# Autodesk Inventor assembly: ASY GBK 3110 central wall shield 1
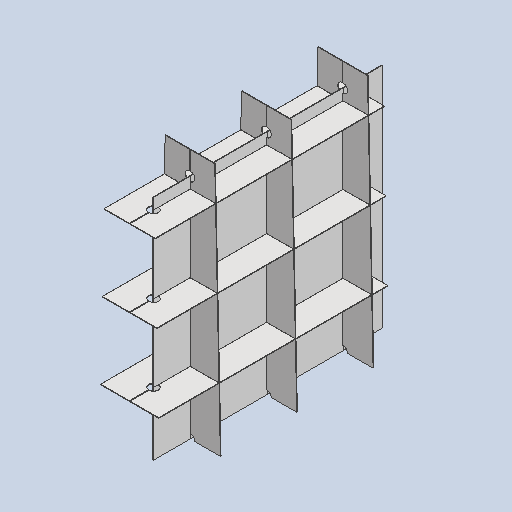
[picture p0: Inventor's stored thumbnail of the model, 512x512]
Saved by Autodesk Inventor 2026 (Build 300175000, 175)
## iProperties
Created: 2026-05-19
Part Number: ASY GBK 3110 central wall shield 1
Document SubType Name: Assembly
Designer: pokla
Mass: 174041 g
Surface Area: 113034 cm^2
Volume: 22170.8 cm^3
Density: 7.85 g/cm^3
Author: admin
## Documents named in this file (7)
- C:\Users\pokla\Documents\Inventor\GBK-Gubkinskiy\ASY GBK 3110 central wall shield 1.iam
- C:\Users\pokla\Documents\Inventor\GBK-Gubkinskiy\GBK 3113 stringer 1.ipt
- C:\Users\pokla\Documents\Inventor\GBK-Gubkinskiy\GBK 3111 shield 1.ipt
- C:\Users\pokla\Documents\Inventor\GBK-Gubkinskiy\GBK 3114 stringer 2.ipt
- C:\Users\pokla\Documents\Inventor\GBK-Gubkinskiy\GBK 3115 stringer 3.ipt
- C:\Users\pokla\Documents\Inventor\GBK-Gubkinskiy\GBK 3112 central main rib.ipt
- C:\Users\pokla\Documents\Inventor\GBK-Gubkinskiy\GBK 0101 main rib.ipt
## Components (13 placed, 8 different names)
1. GBK 3113 stringer 1.ipt:1 — Жесткий:1
2. GBK 3111 shield 1.ipt:1 — Заподлицо:5, Совмещение:5, Заподлицо:3, Совмещение:2, Заподлицо:1, Совмещение:1, Совмещение:4, Заподлицо:2
3. GBK 3114 stringer 2.ipt:1 — Жесткий:2
4. GBK 3115 stringer 3.ipt:1 — Жесткий:3
5. GBK 3113 stringer 1.ipt:2 — Жесткий:6
6. GBK 3114 stringer 2:3 — Жесткий:5
7. GBK 3115 stringer 3:2 — Жесткий:6
8. GBK 3112 central main rib.ipt:2 — Заподлицо:4, Совмещение:4, Заподлицо:2, Жесткий:6, Жесткий:5, Жесткий:6
9. GBK 3112 central main rib:3
10. GBK 3112 central main rib:4
11. GBK 3112 central main rib.ipt:1 — Заподлицо:5, Совмещение:5, Заподлицо:3, Заподлицо:4, Жесткий:1, Жесткий:2, Жесткий:3
12. GBK 3112 central main rib:5
13. GBK 3112 central main rib:6
## Component patterns: (3 elements, first: GBK 3112 central main rib.ipt:2), (3 elements, first: GBK 3112 central main rib.ipt:1)
## Relationships (15: WeldJoint 6, Flush 5, Mate 4)
- Заподлицо:5 [Flush] (254 mm): GBK 3111 shield 1.ipt:1 ↔ GBK 3112 central main rib.ipt:1
- Совмещение:5 [Mate]: GBK 3111 shield 1.ipt:1 ↔ GBK 3112 central main rib.ipt:1
- Заподлицо:3 [Flush]: GBK 3111 shield 1.ipt:1 ↔ GBK 3112 central main rib.ipt:1
- Совмещение:2 [Mate]: GBK 3111 shield 1.ipt:1
- Заподлицо:1 [Flush]: GBK 3111 shield 1.ipt:1
- Совмещение:1 [Mate]: GBK 3111 shield 1.ipt:1
- Заподлицо:4 [Flush]: GBK 3112 central main rib.ipt:2 ↔ GBK 3112 central main rib.ipt:1
- Совмещение:4 [Mate]: GBK 3111 shield 1.ipt:1 ↔ GBK 3112 central main rib.ipt:2
- Заподлицо:2 [Flush]: GBK 3111 shield 1.ipt:1 ↔ GBK 3112 central main rib.ipt:2
- Жесткий:1 [WeldJoint] (4 mm): GBK 3113 stringer 1.ipt:1 ↔ GBK 3112 central main rib.ipt:1
- Жесткий:2 [WeldJoint] (4 mm): GBK 3114 stringer 2.ipt:1 ↔ GBK 3112 central main rib.ipt:1
- Жесткий:3 [WeldJoint] (4 mm): GBK 3115 stringer 3.ipt:1 ↔ GBK 3112 central main rib.ipt:1
- Жесткий:6 [WeldJoint] (4 mm): GBK 3113 stringer 1.ipt:2 ↔ GBK 3112 central main rib.ipt:2
- Жесткий:5 [WeldJoint] (4 mm): GBK 3114 stringer 2:3 ↔ GBK 3112 central main rib.ipt:2
- Жесткий:6 [WeldJoint] (4 mm): GBK 3115 stringer 3:2 ↔ GBK 3112 central main rib.ipt:2
## Named parameters: Шаг_шпангоутов = 496.66667 mm
